# Autodesk Inventor assembly: assemble_ver5_prod_sector2
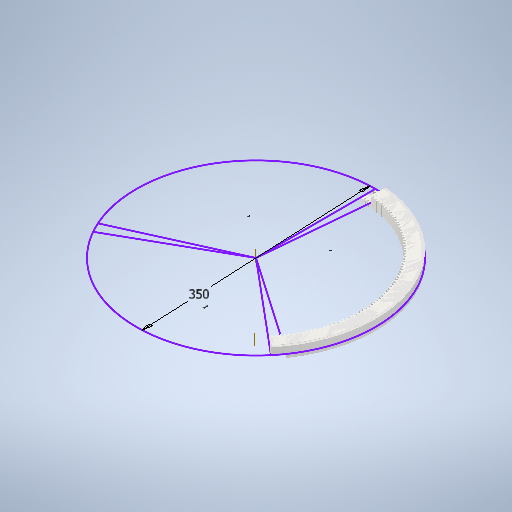
[picture p0: Inventor's stored thumbnail of the model, 512x512]
Saved by Autodesk Inventor 2025 (Build 290162000, 162)
## iProperties
Created: 2025-12-09
Part Number: assemble_ver5_prod_sector2
Document SubType Name: Assembly
Designer: Admin
Author: Admin
## Documents named in this file (2)
- C:\Users\sum89\OneDrive\Рабочий стол\Ring\Model\assemble_ver5_prod_sector2.iam
- C:\Users\sum89\OneDrive\Рабочий стол\Ring\Model\assemble_ver5_thick.iam
## Components (1 placed, 1 different names)
1. assemble_ver5_thick:1 [sub-assembly] — Совмещение:1, Совмещение:2
## Relationships (2: Mate 2)
- Совмещение:1 [Mate]: assemble_ver5_thick:1
- Совмещение:2 [Mate]: assemble_ver5_thick:1
